# Autodesk Inventor assembly: footprint_placement
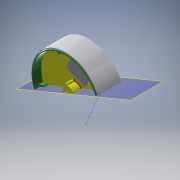
[picture p0: Inventor's stored thumbnail of the model, 180x180]
Saved by Autodesk Inventor 2019 (Build 230136000, 136)
## iProperties
Created: 2019-04-10
Part Number: footprint_placement
Document SubType Name: Assembly
Designer: jmc
Author: jmc
## Documents named in this file (5)
- C:\Users\l0086\Desktop\Models\CatFeeder\Case\version6\footprint_placement.iam
- C:\Users\l0086\Desktop\Models\CatFeeder\Case\version6\wheel8.ipt
- C:\Users\l0086\Desktop\Models\CatFeeder\Case\version6\esp8266_footprint.ipt
- C:\Users\l0086\Desktop\Models\CatFeeder\Case\version6\motordriver_footprint.ipt
- C:\Users\l0086\Desktop\Models\CatFeeder\Case\version6\separator.ipt
## Components (4 placed, 4 different names)
1. wheel8:1 — Rigid:3
2. esp8266_footprint:1 — Rotational:1
3. motordriver_footprint:1
4. separator:1 — Rigid:3, Rotational:1
## Relationships (2: WeldJoint 1, RevoluteJoint 1)
- Rigid:3 [WeldJoint]: wheel8:1 ↔ separator:1
- Rotational:1 [RevoluteJoint]: esp8266_footprint:1 ↔ separator:1
